# Autodesk Inventor assembly: HERA_NODE_ENCLOSURE_ASSEMBLY
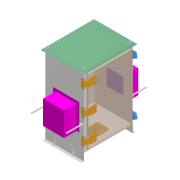
[picture p0: Inventor's stored thumbnail of the model, 180x180]
Saved by Autodesk Inventor 2017 (Build 210142000, 142)
## iProperties
Created: 2018-10-04
Part Number: HERA_NODE_ENCLOSURE_ASSEMBLY
Document SubType Name: Assembly
Designer: Kathryn Rosie
Sending System: Autodesk Inventor 2018
Preprocessor: ST-DEVELOPER v16.13
Title: D:\ITC\DRAWINGS\SKA PROJECT\HERA NODE\HERA NODE 2018 TENDER SUBMISIONS\ASSEMBLY\HERA_NODE_ENCLOSURE_ASSEMBLY.stp
Author: Francois
## Documents named in this file (21)
- C:\Users\Kathryn Rosie\Google Drive\HERA\Node\4. Concept Design\HERA_NODE_ENCLOSURE_ASSEMBLY.iam
- C:\Users\Kathryn Rosie\Google Drive\HERA\Node\4. Concept Design\HERA_NODE_BOTTOM_PLATE.ipt
- C:\Users\Kathryn Rosie\Google Drive\HERA\Node\4. Concept Design\HERA_NODE_LEFT_SIDE_PLATE.ipt
- C:\Users\Kathryn Rosie\Google Drive\HERA\Node\4. Concept Design\HERA_NODE_RIGHT_SIDE_PLATE.ipt
- C:\Users\Kathryn Rosie\Google Drive\HERA\Node\4. Concept Design\HERA_NODE_TOP_PLATE.ipt
- C:\Users\Kathryn Rosie\Google Drive\HERA\Node\4. Concept Design\HERA_NODE_BACK_PLATE.ipt
- C:\Users\Kathryn Rosie\Google Drive\HERA\Node\4. Concept Design\HERA_NODE_FOOTPLATE_ASSEMBLY.iam
- C:\Users\Kathryn Rosie\Google Drive\HERA\Node\4. Concept Design\HERA_NODE_DOOR_ASSEMBLY.iam
- C:\Users\Kathryn Rosie\Google Drive\HERA\Node\4. Concept Design\FILTER_PLATE_RP.ipt
- C:\Users\Kathryn Rosie\Google Drive\HERA\Node\4. Concept Design\FILTER_PLATE_LP.ipt
- C:\Users\Kathryn Rosie\Google Drive\HERA\Node\4. Concept Design\TOP_VENT.ipt
- C:\Users\Kathryn Rosie\Google Drive\HERA\Node\4. Concept Design\BOTTOM_VENT.ipt
- C:\Users\Kathryn Rosie\Google Drive\HERA\Node\4. Concept Design\HINGE_ASSEMBLY.iam
- C:\Users\Kathryn Rosie\Google Drive\HERA\Node\4. Concept Design\FILTER_PANEL_COVER_RP.ipt
- C:\Users\Kathryn Rosie\Google Drive\HERA\Node\4. Concept Design\LIFTING_LUG_SUPPORT.ipt
- C:\Users\Kathryn Rosie\Google Drive\HERA\Node\4. Concept Design\ROOF_PANEL.ipt
- C:\Users\Kathryn Rosie\Google Drive\HERA\Node\4. Concept Design\LIFTING_LUG.ipt
- C:\Users\Kathryn Rosie\Google Drive\HERA\Node\4. Concept Design\CARRY_HANDLE_SUPPORT.ipt
- C:\Users\Kathryn Rosie\Google Drive\HERA\Node\4. Concept Design\CARRY_HANDLE.ipt
- C:\Users\Kathryn Rosie\Google Drive\HERA\Node\4. Concept Design\DOOR_LOCK_CATCH.ipt
- C:\Users\Kathryn Rosie\Google Drive\HERA\hera-cad-0\Node\Tender Model\nodeContents.iam
## Components (37 placed, 20 different names)
1. HERA_NODE_BOTTOM_PLATE:1 — Mate:4, Mate:5, Mate:6, Mate:7, Mate:8, Mate:9, Mate:10, Mate:12, Mate:59, Mate:60, Mate:61, Flush:23, Mate:76
2. HERA_NODE_LEFT_SIDE_PLATE:1 — Mate:2, Mate:3, Mate:12, Mate:13, Flush:2, Mate:18, Mate:19, Flush:10, Mate:33, Mate:34, Mate:35, Mate:36, Tangent:1, Mate:38, Mate:39, Tangent:2, Mate:40, Mate:41, Tangent:3, Flush:14, Flush:15, Flush:16, Mate:49, Flush:18
3. HERA_NODE_RIGHT_SIDE_PLATE:1 — Mate:10, Mate:11, Flush:1, Mate:14, Flush:4, Mate:15, Flush:5, Mate:17, Mate:28, Mate:29, Mate:30, Mate:32, Flush:20, Flush:21, Flush:22, Mate:62, Mate:63, Mate:64, Mate:65
4. HERA_NODE_TOP_PLATE:1 — Mate:42, Mate:45, Mate:48, Mate:49, Flush:18, Mate:50, Mate:53, Mate:56, Mate:57, Mate:58, Flush:24
5. HERA_NODE_BACK_PLATE:1 — Mate:15, Mate:16, Flush:5, Flush:6, Flush:8, Flush:17, Mate:48, Flush:19
6. HERA_NODE_FOOTPLATE_ASSEMBLY:1 [sub-assembly] — Mate:4, Mate:5, Mate:6, Mate:13, Flush:2, Flush:9, Flush:11
7. HERA_NODE_FOOTPLATE_ASSEMBLY:2 [sub-assembly] — Mate:7, Mate:8, Mate:9, Mate:11, Flush:1, Flush:3, Mate:16, Flush:7
8. HERA_NODE_DOOR_ASSEMBLY:1 [sub-assembly] — Mate:74, Tangent:4, Tangent:5, Mate:75
9. FILTER_PLATE_RP:1 — Mate:28, Mate:29, Mate:30, Mate:31, Flush:12
10. FILTER_PLATE_LP:1 — Mate:33, Mate:34, Mate:35, Mate:37, Flush:13
11. TOP_VENT:1 — Mate:56, Mate:57, Mate:58
12. BOTTOM_VENT:1 — Mate:59, Mate:60, Mate:61, Mate:77
13. HINGE_ASSEMBLY:1 [sub-assembly] — Mate:40, Mate:41, Tangent:3, Mate:75
14. HINGE_ASSEMBLY:2 [sub-assembly] — Mate:2, Mate:3, Tangent:1, Mate:74, Tangent:4
15. HINGE_ASSEMBLY:3 [sub-assembly] — Mate:38, Mate:39, Tangent:2, Tangent:5
16. FILTER_PANEL_COVER_RP:1 — Mate:31, Flush:12, Mate:32
17. FILTER_PANEL_COVER_RP:2 — Mate:36, Mate:37, Flush:13
18. LIFTING_LUG_SUPPORT:1 — Flush:14, Flush:15, Mate:42, Mate:43, Angle:5, Mate:66, Mate:68
19. LIFTING_LUG_SUPPORT:2 — Mate:53, Flush:21, Flush:22, Mate:54, Angle:8
20. LIFTING_LUG_SUPPORT:3 — Mate:45, Flush:16, Flush:17, Mate:46, Angle:6, Mate:67
21. LIFTING_LUG_SUPPORT:4 — Mate:50, Flush:19, Flush:20, Angle:7, Mate:69
22. ROOF_PANEL:1 — Mate:66, Mate:67, Mate:68, Mate:70, Mate:71, Mate:72, Mate:73
23. LIFTING_LUG:1 — Mate:43, Angle:5, Mate:71
24. LIFTING_LUG:2 — Mate:46, Angle:6, Mate:73
25. LIFTING_LUG:3 — Mate:54, Angle:8, Mate:72
26. LIFTING_LUG:4 — Angle:7, Mate:69, Mate:70
27. CARRY_HANDLE_SUPPORT:1 — Mate:19, Flush:10, Flush:11, Mate:22, Mate:23, Angle:2
28. CARRY_HANDLE_SUPPORT:2 — Mate:18, Flush:8, Flush:9, Mate:20, Mate:21, Angle:1
29. CARRY_HANDLE_SUPPORT:3 — Mate:17, Flush:6, Flush:7, Mate:26, Mate:27, Angle:4
30. CARRY_HANDLE_SUPPORT:4 — Mate:14, Flush:3, Flush:4, Mate:24, Mate:25, Angle:3
31. CARRY_HANDLE:1 — Mate:26, Mate:27, Angle:4
32. CARRY_HANDLE:2 — Mate:24, Mate:25, Angle:3
33. CARRY_HANDLE:3 — Mate:20, Mate:21, Angle:1
34. CARRY_HANDLE:4 — Mate:22, Mate:23, Angle:2
35. DOOR_LOCK_CATCH:1 — Flush:24, Mate:62, Mate:63
36. DOOR_LOCK_CATCH:2 — Flush:23, Mate:64, Mate:65
37. nodeContents:1 [sub-assembly] — Mate:76, Mate:77
## Relationships (108: Mate 71, Flush 24, Angle 8, Tangent 5)
- Mate:2: HERA_NODE_LEFT_SIDE_PLATE:1 ↔ HINGE_ASSEMBLY:2
- Mate:3: HERA_NODE_LEFT_SIDE_PLATE:1 ↔ HINGE_ASSEMBLY:2
- Mate:4: HERA_NODE_BOTTOM_PLATE:1 ↔ HERA_NODE_FOOTPLATE_ASSEMBLY:1
- Mate:5: HERA_NODE_BOTTOM_PLATE:1 ↔ HERA_NODE_FOOTPLATE_ASSEMBLY:1
- Mate:6: HERA_NODE_BOTTOM_PLATE:1 ↔ HERA_NODE_FOOTPLATE_ASSEMBLY:1
- Mate:7: HERA_NODE_BOTTOM_PLATE:1 ↔ HERA_NODE_FOOTPLATE_ASSEMBLY:2
- Mate:8: HERA_NODE_BOTTOM_PLATE:1 ↔ HERA_NODE_FOOTPLATE_ASSEMBLY:2
- Mate:9: HERA_NODE_BOTTOM_PLATE:1 ↔ HERA_NODE_FOOTPLATE_ASSEMBLY:2
- Mate:10: HERA_NODE_BOTTOM_PLATE:1 ↔ HERA_NODE_RIGHT_SIDE_PLATE:1
- Mate:11: HERA_NODE_RIGHT_SIDE_PLATE:1 ↔ HERA_NODE_FOOTPLATE_ASSEMBLY:2
- Flush:1: HERA_NODE_RIGHT_SIDE_PLATE:1 ↔ HERA_NODE_FOOTPLATE_ASSEMBLY:2
- Mate:12: HERA_NODE_BOTTOM_PLATE:1 ↔ HERA_NODE_LEFT_SIDE_PLATE:1
- Mate:13: HERA_NODE_LEFT_SIDE_PLATE:1 ↔ HERA_NODE_FOOTPLATE_ASSEMBLY:1
- Flush:2: HERA_NODE_LEFT_SIDE_PLATE:1 ↔ HERA_NODE_FOOTPLATE_ASSEMBLY:1
- Mate:14: HERA_NODE_RIGHT_SIDE_PLATE:1 ↔ CARRY_HANDLE_SUPPORT:4
- Flush:3 (600 mm): HERA_NODE_FOOTPLATE_ASSEMBLY:2 ↔ CARRY_HANDLE_SUPPORT:4
- Flush:4 (20 mm): HERA_NODE_RIGHT_SIDE_PLATE:1 ↔ CARRY_HANDLE_SUPPORT:4
- Mate:15: HERA_NODE_RIGHT_SIDE_PLATE:1 ↔ HERA_NODE_BACK_PLATE:1
- Mate:16: HERA_NODE_BACK_PLATE:1 ↔ HERA_NODE_FOOTPLATE_ASSEMBLY:2
- Flush:5: HERA_NODE_RIGHT_SIDE_PLATE:1 ↔ HERA_NODE_BACK_PLATE:1
- Mate:17: HERA_NODE_RIGHT_SIDE_PLATE:1 ↔ CARRY_HANDLE_SUPPORT:3
- Flush:6 (20 mm): HERA_NODE_BACK_PLATE:1 ↔ CARRY_HANDLE_SUPPORT:3
- Flush:7 (600 mm): HERA_NODE_FOOTPLATE_ASSEMBLY:2 ↔ CARRY_HANDLE_SUPPORT:3
- Mate:18: HERA_NODE_LEFT_SIDE_PLATE:1 ↔ CARRY_HANDLE_SUPPORT:2
- Flush:8 (20 mm): HERA_NODE_BACK_PLATE:1 ↔ CARRY_HANDLE_SUPPORT:2
- Flush:9 (600 mm): HERA_NODE_FOOTPLATE_ASSEMBLY:1 ↔ CARRY_HANDLE_SUPPORT:2
- Mate:19: HERA_NODE_LEFT_SIDE_PLATE:1 ↔ CARRY_HANDLE_SUPPORT:1
- Flush:10 (20 mm): HERA_NODE_LEFT_SIDE_PLATE:1 ↔ CARRY_HANDLE_SUPPORT:1
- Flush:11 (600 mm): HERA_NODE_FOOTPLATE_ASSEMBLY:1 ↔ CARRY_HANDLE_SUPPORT:1
- Mate:20: CARRY_HANDLE_SUPPORT:2 ↔ CARRY_HANDLE:3
- Mate:21: CARRY_HANDLE_SUPPORT:2 ↔ CARRY_HANDLE:3
- Angle:1 (0 deg): CARRY_HANDLE_SUPPORT:2 ↔ CARRY_HANDLE:3
- Mate:22: CARRY_HANDLE_SUPPORT:1 ↔ CARRY_HANDLE:4
- Mate:23: CARRY_HANDLE_SUPPORT:1 ↔ CARRY_HANDLE:4
- Angle:2 (0 deg): CARRY_HANDLE_SUPPORT:1 ↔ CARRY_HANDLE:4
- Mate:24: CARRY_HANDLE_SUPPORT:4 ↔ CARRY_HANDLE:2
- Mate:25: CARRY_HANDLE_SUPPORT:4 ↔ CARRY_HANDLE:2
- Angle:3 (0 deg): CARRY_HANDLE_SUPPORT:4 ↔ CARRY_HANDLE:2
- Mate:26: CARRY_HANDLE_SUPPORT:3 ↔ CARRY_HANDLE:1
- Mate:27: CARRY_HANDLE_SUPPORT:3 ↔ CARRY_HANDLE:1
- Angle:4 (0 deg): CARRY_HANDLE_SUPPORT:3 ↔ CARRY_HANDLE:1
- Mate:28: HERA_NODE_RIGHT_SIDE_PLATE:1 ↔ FILTER_PLATE_RP:1
- Mate:29: HERA_NODE_RIGHT_SIDE_PLATE:1 ↔ FILTER_PLATE_RP:1
- Mate:30: HERA_NODE_RIGHT_SIDE_PLATE:1 ↔ FILTER_PLATE_RP:1
- Mate:31 (3 mm): FILTER_PLATE_RP:1 ↔ FILTER_PANEL_COVER_RP:1
- Flush:12 (-55 mm): FILTER_PLATE_RP:1 ↔ FILTER_PANEL_COVER_RP:1
- Mate:32: HERA_NODE_RIGHT_SIDE_PLATE:1 ↔ FILTER_PANEL_COVER_RP:1
- Mate:33: HERA_NODE_LEFT_SIDE_PLATE:1 ↔ FILTER_PLATE_LP:1
- Mate:34: HERA_NODE_LEFT_SIDE_PLATE:1 ↔ FILTER_PLATE_LP:1
- Mate:35: HERA_NODE_LEFT_SIDE_PLATE:1 ↔ FILTER_PLATE_LP:1
- Mate:36: HERA_NODE_LEFT_SIDE_PLATE:1 ↔ FILTER_PANEL_COVER_RP:2
- Mate:37 (3 mm): FILTER_PLATE_LP:1 ↔ FILTER_PANEL_COVER_RP:2
- Flush:13 (55 mm): FILTER_PLATE_LP:1 ↔ FILTER_PANEL_COVER_RP:2
- Tangent:1 (0.5 mm): HERA_NODE_LEFT_SIDE_PLATE:1 ↔ HINGE_ASSEMBLY:2
- Mate:38: HERA_NODE_LEFT_SIDE_PLATE:1 ↔ HINGE_ASSEMBLY:3
- Mate:39: HERA_NODE_LEFT_SIDE_PLATE:1 ↔ HINGE_ASSEMBLY:3
- Tangent:2 (0.5 mm): HERA_NODE_LEFT_SIDE_PLATE:1 ↔ HINGE_ASSEMBLY:3
- Mate:40: HERA_NODE_LEFT_SIDE_PLATE:1 ↔ HINGE_ASSEMBLY:1
- Mate:41: HERA_NODE_LEFT_SIDE_PLATE:1 ↔ HINGE_ASSEMBLY:1
- Tangent:3 (0.5 mm): HERA_NODE_LEFT_SIDE_PLATE:1 ↔ HINGE_ASSEMBLY:1
- Flush:14 (7 mm): HERA_NODE_LEFT_SIDE_PLATE:1 ↔ LIFTING_LUG_SUPPORT:1
- Flush:15 (7 mm): HERA_NODE_LEFT_SIDE_PLATE:1 ↔ LIFTING_LUG_SUPPORT:1
- Mate:42: HERA_NODE_TOP_PLATE:1 ↔ LIFTING_LUG_SUPPORT:1
- Mate:43: LIFTING_LUG_SUPPORT:1 ↔ LIFTING_LUG:1
- Angle:5 (0 deg): LIFTING_LUG_SUPPORT:1 ↔ LIFTING_LUG:1
- Mate:45: HERA_NODE_TOP_PLATE:1 ↔ LIFTING_LUG_SUPPORT:3
- Flush:16 (7 mm): HERA_NODE_LEFT_SIDE_PLATE:1 ↔ LIFTING_LUG_SUPPORT:3
- Flush:17 (7 mm): HERA_NODE_BACK_PLATE:1 ↔ LIFTING_LUG_SUPPORT:3
- Mate:46: LIFTING_LUG_SUPPORT:3 ↔ LIFTING_LUG:2
- Angle:6 (0 deg): LIFTING_LUG_SUPPORT:3 ↔ LIFTING_LUG:2
- Mate:48: HERA_NODE_TOP_PLATE:1 ↔ HERA_NODE_BACK_PLATE:1
- Mate:49: HERA_NODE_LEFT_SIDE_PLATE:1 ↔ HERA_NODE_TOP_PLATE:1
- Flush:18: HERA_NODE_LEFT_SIDE_PLATE:1 ↔ HERA_NODE_TOP_PLATE:1
- Mate:50: HERA_NODE_TOP_PLATE:1 ↔ LIFTING_LUG_SUPPORT:4
- Flush:19 (7 mm): HERA_NODE_BACK_PLATE:1 ↔ LIFTING_LUG_SUPPORT:4
- Flush:20 (7 mm): HERA_NODE_RIGHT_SIDE_PLATE:1 ↔ LIFTING_LUG_SUPPORT:4
- Angle:7 (0 deg): LIFTING_LUG_SUPPORT:4 ↔ LIFTING_LUG:4
- Mate:53: HERA_NODE_TOP_PLATE:1 ↔ LIFTING_LUG_SUPPORT:2
- Flush:21 (7 mm): HERA_NODE_RIGHT_SIDE_PLATE:1 ↔ LIFTING_LUG_SUPPORT:2
- Flush:22 (7 mm): HERA_NODE_RIGHT_SIDE_PLATE:1 ↔ LIFTING_LUG_SUPPORT:2
- Mate:54: LIFTING_LUG_SUPPORT:2 ↔ LIFTING_LUG:3
- Angle:8 (0 deg): LIFTING_LUG_SUPPORT:2 ↔ LIFTING_LUG:3
- Mate:56: HERA_NODE_TOP_PLATE:1 ↔ TOP_VENT:1
- Mate:57: HERA_NODE_TOP_PLATE:1 ↔ TOP_VENT:1
- Mate:58: HERA_NODE_TOP_PLATE:1 ↔ TOP_VENT:1
- Mate:59: HERA_NODE_BOTTOM_PLATE:1 ↔ BOTTOM_VENT:1
- Mate:60: HERA_NODE_BOTTOM_PLATE:1 ↔ BOTTOM_VENT:1
- Mate:61: HERA_NODE_BOTTOM_PLATE:1 ↔ BOTTOM_VENT:1
- Flush:23 (100 mm): HERA_NODE_BOTTOM_PLATE:1 ↔ DOOR_LOCK_CATCH:2
- Flush:24 (100 mm): HERA_NODE_TOP_PLATE:1 ↔ DOOR_LOCK_CATCH:1
- Mate:62: HERA_NODE_RIGHT_SIDE_PLATE:1 ↔ DOOR_LOCK_CATCH:1
- Mate:63: HERA_NODE_RIGHT_SIDE_PLATE:1 ↔ DOOR_LOCK_CATCH:1
- Mate:64: HERA_NODE_RIGHT_SIDE_PLATE:1 ↔ DOOR_LOCK_CATCH:2
- Mate:65: HERA_NODE_RIGHT_SIDE_PLATE:1 ↔ DOOR_LOCK_CATCH:2
- Mate:66: LIFTING_LUG_SUPPORT:1 ↔ ROOF_PANEL:1
- Mate:67: LIFTING_LUG_SUPPORT:3 ↔ ROOF_PANEL:1
- Mate:68: LIFTING_LUG_SUPPORT:1 ↔ ROOF_PANEL:1
- Mate:69: LIFTING_LUG_SUPPORT:4 ↔ LIFTING_LUG:4
- Mate:70: ROOF_PANEL:1 ↔ LIFTING_LUG:4
- Mate:71: ROOF_PANEL:1 ↔ LIFTING_LUG:1
- Mate:72: ROOF_PANEL:1 ↔ LIFTING_LUG:3
- Mate:73: ROOF_PANEL:1 ↔ LIFTING_LUG:2
- Mate:74: HERA_NODE_DOOR_ASSEMBLY:1 ↔ HINGE_ASSEMBLY:2
- Tangent:4 (0.5 mm): HERA_NODE_DOOR_ASSEMBLY:1 ↔ HINGE_ASSEMBLY:2
- Tangent:5 (0.5 mm): HERA_NODE_DOOR_ASSEMBLY:1 ↔ HINGE_ASSEMBLY:3
- Mate:75 (7.5 mm): HERA_NODE_DOOR_ASSEMBLY:1 ↔ HINGE_ASSEMBLY:1
- Mate:76: HERA_NODE_BOTTOM_PLATE:1 ↔ nodeContents:1
- Mate:77: BOTTOM_VENT:1 ↔ nodeContents:1
